# Autodesk Inventor assembly: EnsambleResistencia
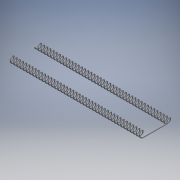
[picture p0: Inventor's stored thumbnail of the model, 180x180]
Saved by Autodesk Inventor 2017 (Build 210142000, 142)
## iProperties
Created: 2021-02-15
Part Number: EnsambleResistencia
Document SubType Name: Assembly
Designer: USUARIO
Author: USUARIO
## Documents named in this file (3)
- D:\Laboratorio\Mufla\2021\Mufla 4.5L Psoc MYC Lab #0045885XX OP202145\Modelo\EnsambleResistencia.iam
- D:\Laboratorio\Mufla\2021\Mufla 4.5L Psoc MYC Lab #0045885XX OP202145\Modelo\Resistencia.ipt
- D:\Laboratorio\Mufla\2021\Mufla 4.5L Psoc MYC Lab #0045885XX OP202145\Modelo\Resistencia2.ipt
## Components (2 placed, 2 different names)
1. Resistencia:1 — Tangent:1
2. Resistencia2:1 — Tangent:1
## Relationships (1: Tangent 1)
- Tangent:1: Resistencia:1 ↔ Resistencia2:1
